# Autodesk Inventor assembly: CG_Maschine
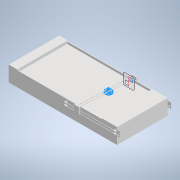
[picture p0: Inventor's stored thumbnail of the model, 180x180]
Saved by Autodesk Inventor 2021 (Build 250183000, 183)
## iProperties
Created: 2021-05-21
Part Number: CG_Maschine
Document SubType Name: Assembly
Designer: marce
Author: marce
## Documents named in this file (10)
- C:\Users\marce\Documents\Autodesk Projekte\CG_Maschine.iam
- C:\Users\marce\Documents\Autodesk Projekte\Tisch.ipt
- C:\Users\marce\Downloads\YAchseBasisteil-2.ipt
- C:\Users\marce\Downloads\HalterungMotorNeu(1).ipt
- C:\Users\marce\Downloads\HalterungMotorNeuAndereSeite.ipt
- C:\Users\marce\Downloads\HalterungStangeNeu(1).ipt
- C:\Users\marce\Documents\Autodesk Projekte\KI_Pusher.ipt
- C:\Users\marce\Documents\Autodesk Projekte\Stange.ipt
- C:\Users\marce\Documents\Autodesk Projekte\StangeY.ipt
- C:\Users\marce\Documents\Autodesk Projekte\Linearlager.ipt
## Components (16 placed, 9 different names)
1. Tisch:1 — Passend:1, Passend:2, Passend:3, Passend:4, Passend:5
2. YAchseBasisteil-2:1 — Einfügen:9, Einfügen:10
3. HalterungMotorNeu(1):2 — Passend:3, Einfügen:5
4. HalterungMotorNeuAndereSeite:1 — Passend:1, Einfügen:6
5. HalterungStangeNeu(1):1 — Passend:4, Einfügen:3, Einfügen:4
6. HalterungStangeNeu(1):2 — Passend:2, Einfügen:1, Einfügen:2
7. YAchseBasisteil-2:2 — Einfügen:7, Einfügen:8
8. KI_Pusher:1 — Passend:5, Passend:6, Passend:7
9. Stange:1 — Einfügen:1
10. Stange:2 — Einfügen:3
11. Stange:3 — Einfügen:4, Einfügen:5
12. Stange:4 — Einfügen:2, Einfügen:6
13. StangeY:1 — Einfügen:8, Einfügen:9, Passend:8
14. StangeY:2 — Einfügen:7, Einfügen:10
15. Linearlager:4 — Passend:7
16. Linearlager:6 — Passend:6, Passend:8
## Relationships (18: Insert 10, Mate 8)
- Passend:1 [Mate]: Tisch:1 ↔ HalterungMotorNeuAndereSeite:1
- Passend:2 [Mate]: Tisch:1 ↔ HalterungStangeNeu(1):2
- Passend:3 [Mate]: Tisch:1 ↔ HalterungMotorNeu(1):2
- Passend:4 [Mate]: Tisch:1 ↔ HalterungStangeNeu(1):1
- Passend:5 [Mate] (5 mm): Tisch:1 ↔ KI_Pusher:1
- Einfügen:1 [Insert]: HalterungStangeNeu(1):2 ↔ Stange:1
- Einfügen:2 [Insert]: HalterungStangeNeu(1):2 ↔ Stange:4
- Einfügen:3 [Insert]: HalterungStangeNeu(1):1 ↔ Stange:2
- Einfügen:4 [Insert]: HalterungStangeNeu(1):1 ↔ Stange:3
- Einfügen:5 [Insert]: HalterungMotorNeu(1):2 ↔ Stange:3
- Einfügen:6 [Insert]: HalterungMotorNeuAndereSeite:1 ↔ Stange:4
- Einfügen:7 [Insert]: YAchseBasisteil-2:2 ↔ StangeY:2
- Einfügen:8 [Insert]: YAchseBasisteil-2:2 ↔ StangeY:1
- Einfügen:9 [Insert]: YAchseBasisteil-2:1 ↔ StangeY:1
- Einfügen:10 [Insert]: YAchseBasisteil-2:1 ↔ StangeY:2
- Passend:6 [Mate]: KI_Pusher:1 ↔ Linearlager:6
- Passend:7 [Mate]: KI_Pusher:1 ↔ Linearlager:4
- Passend:8 [Mate]: StangeY:1 ↔ Linearlager:6
